# Autodesk Inventor assembly: Front Hub Carrier R
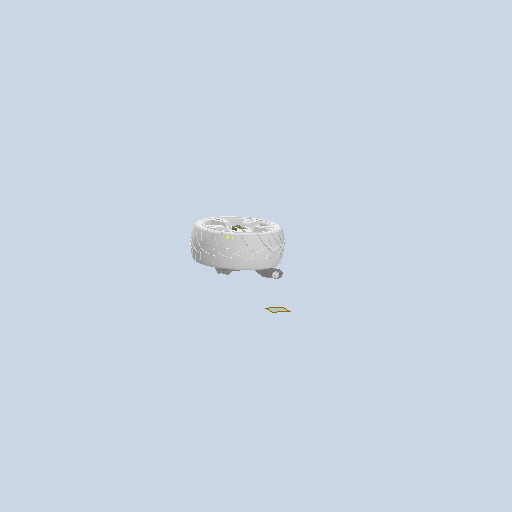
[picture p0: Inventor's stored thumbnail of the model, 512x512]
Saved by Autodesk Inventor 2024 (Build 280153000, 153)
## iProperties
Created: 2023-07-07
Part Number: Front Hub Carrier R
Document SubType Name: Assembly
Designer: birud
Author: birud
## Documents named in this file (14)
- C:\Users\_Astitva_Aryan_\Downloads\ES101_Components_Group5\Components_derived\Front Hub Carrier R.iam
- C:\Users\_Astitva_Aryan_\Downloads\ES101_Components_Group5\Components_derived\Front hub carrier R.ipt
- C:\Users\_Astitva_Aryan_\Downloads\ES101_Components_Group5\Components_derived\Pillow Ball Retainer-1.ipt
- C:\Users\_Astitva_Aryan_\Downloads\ES101_Components_Group5\Components_derived\Pillow Ball Bushing.ipt
- C:\Users\_Astitva_Aryan_\Downloads\ES101_Components_Group5\Components_derived\rear hub bearing.ipt
- C:\Users\_Astitva_Aryan_\Downloads\ES101_Components_Group5\Components_derived\front hub bearing.ipt
- C:\Users\_Astitva_Aryan_\Downloads\ES101_Components_Group5\Components_derived\front axle.ipt
- C:\Users\_Astitva_Aryan_\Downloads\ES101_Components_Group5\Components_derived\Ball Stud.ipt
- C:\Users\_Astitva_Aryan_\Downloads\ES101_Components_Group5\Components_derived\HexDrive.ipt
- C:\Users\_Astitva_Aryan_\Downloads\ES101_Components_Group5\Components_derived\hex retaining o-ring.ipt
- C:\Users\_Astitva_Aryan_\Downloads\ES101_Components_Group5\Components_derived\hex axle pin.ipt
- C:\Users\_Astitva_Aryan_\Downloads\ES101_Components_Group5\Components_derived\Wheel.ipt
- C:\Users\_Astitva_Aryan_\Downloads\ES101_Components_Group5\Components_derived\Tire.ipt
- C:\Users\_Astitva_Aryan_\Downloads\ES101_Components_Group5\Components_derived\ansi.ipt
## Components (15 placed, 13 different names)
1. Front hub carrier R:1 — Mate:1, Mate:2, Flush:1, Flush:2, Mate:3, Mate:4, Mate:7, Flush:3, Mate:8, Flush:4, Mate:10, Insert:1, Mate:18
2. Pillow Ball Retainer-1:1 — Mate:1, Flush:1, Mate:6
3. Pillow Ball Retainer-1:2 — Mate:2, Flush:2, Mate:5
4. Pillow Ball Bushing:1 — Mate:3, Mate:6
5. Pillow Ball Bushing:2 — Mate:4, Mate:5
6. rear hub bearing:1 — Mate:7, Flush:3, Mate:9
7. front hub bearing:1 — Mate:8, Flush:4
8. front axle:1 — Mate:9, Mate:10, Mate:15, Mate:16, Mate:18, Mate:19, Mate:21
9. Ball Stud:1 — Insert:1
10. HexDrive:1 — Mate:11, Mate:12, Mate:13, Mate:14, Mate:15, Mate:20
11. hex retaining o-ring:1 — Mate:13, Flush:5
12. hex axle pin:1 — Mate:11, Mate:12, Mate:16
13. Wheel:1 — Mate:17, Flush:6, Angle:1, Mate:19, Mate:20, Mate:22
14. Tire:1 — Mate:17, Flush:6, Angle:1
15. ansi:1 — Mate:21, Mate:22
## Relationships (30: Mate 22, Flush 6, Insert 1, Angle 1)
- Mate:1: Front hub carrier R:1 ↔ Pillow Ball Retainer-1:1
- Mate:2: Front hub carrier R:1 ↔ Pillow Ball Retainer-1:2
- Flush:1 (38.1 mm): Front hub carrier R:1 ↔ Pillow Ball Retainer-1:1
- Flush:2 (38.1 mm): Front hub carrier R:1 ↔ Pillow Ball Retainer-1:2
- Mate:3: Front hub carrier R:1 ↔ Pillow Ball Bushing:1
- Mate:4: Front hub carrier R:1 ↔ Pillow Ball Bushing:2
- Mate:5: Pillow Ball Retainer-1:2 ↔ Pillow Ball Bushing:2
- Mate:6: Pillow Ball Retainer-1:1 ↔ Pillow Ball Bushing:1
- Mate:7: Front hub carrier R:1 ↔ rear hub bearing:1
- Flush:3: Front hub carrier R:1 ↔ rear hub bearing:1
- Mate:8: Front hub carrier R:1 ↔ front hub bearing:1
- Flush:4: Front hub carrier R:1 ↔ front hub bearing:1
- Mate:9: rear hub bearing:1 ↔ front axle:1
- Mate:10 (142.875 mm): Front hub carrier R:1 ↔ front axle:1
- Insert:1: Front hub carrier R:1 ↔ Ball Stud:1
- Mate:11: HexDrive:1 ↔ hex axle pin:1
- Mate:12: HexDrive:1 ↔ hex axle pin:1
- Mate:13: HexDrive:1 ↔ hex retaining o-ring:1
- Flush:5 (8.001 mm): hex retaining o-ring:1
- Mate:14: HexDrive:1
- Mate:15: front axle:1 ↔ HexDrive:1
- Mate:16: front axle:1 ↔ hex axle pin:1
- Mate:17: Wheel:1 ↔ Tire:1
- Flush:6: Wheel:1 ↔ Tire:1
- Angle:1 (0 deg): Wheel:1 ↔ Tire:1
- Mate:18: Front hub carrier R:1 ↔ front axle:1
- Mate:19: front axle:1 ↔ Wheel:1
- Mate:20: HexDrive:1 ↔ Wheel:1
- Mate:21: front axle:1 ↔ ansi:1
- Mate:22: Wheel:1 ↔ ansi:1
